# Autodesk Inventor assembly: joint4
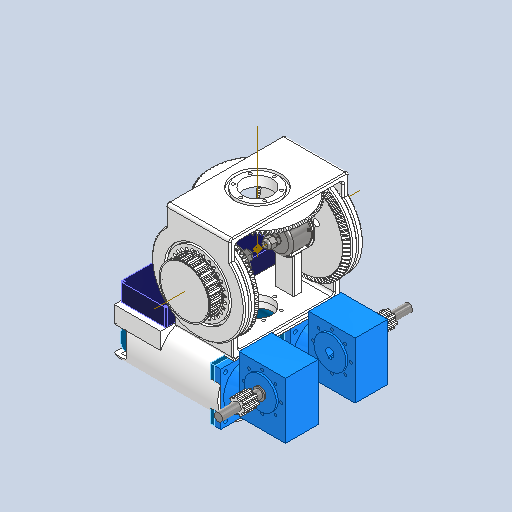
[picture p0: Inventor's stored thumbnail of the model, 512x512]
Saved by Autodesk Inventor 2025.3 (Build 293356030, 356C)
## iProperties
Created: 2025-08-31
Part Number: joint4
Document SubType Name: Assembly
Designer: MSI
Mass: 16930.7 g
Surface Area: 10614.2 cm^2
Volume: 6203.06 cm^3
Density: 2.72942 g/cm^3
Author: MSI
## Documents named in this file (15)
- C:\Users\MSI\Desktop\Project\11. 로봇팔\Robot Arm Model\Robot_Arm_6_v1\joint3.iam
- C:\Users\MSI\Desktop\Project\11. 로봇팔\Robot Arm Model\Robot_Arm_6_v1\motor_holder_1.ipt
- C:\Users\MSI\Desktop\Project\11. 로봇팔\Robot Arm Model\Robot_Arm_6_v1\NMRV30_motor.iam
- C:\Users\MSI\Desktop\Project\11. 로봇팔\Robot Arm Model\Robot_Arm_6_v1\base.ipt
- C:\Users\MSI\Desktop\Project\11. 로봇팔\Robot Arm Model\Robot_Arm_6_v1\frame.ipt
- C:\Users\MSI\Desktop\Project\11. 로봇팔\Robot Arm Model\Robot_Arm_6_v1\miter_gear_center.ipt
- C:\Users\MSI\Desktop\Project\11. 로봇팔\Robot Arm Model\Robot_Arm_6_v1\encoder.ipt
- C:\Users\MSI\Desktop\Project\11. 로봇팔\Robot Arm Model\Robot_Arm_6_v1\belt_pulley_1.ipt
- C:\Users\MSI\Desktop\Project\11. 로봇팔\Robot Arm Model\Robot_Arm_6_v1\belt_pulley_2.ipt
- C:\Users\MSI\Desktop\Project\11. 로봇팔\Robot Arm Model\Robot_Arm_6_v1\motor_shaft.ipt
- C:\Users\MSI\Desktop\Project\11. 로봇팔\Robot Arm Model\Robot_Arm_6_v1\motor_driver.ipt
- C:\Users\MSI\Desktop\Project\11. 로봇팔\Robot Arm Model\Robot_Arm_6_v1\joint3_meteor.iam
- C:\Users\MSI\Desktop\Project\11. 로봇팔\Robot Arm Model\Robot_Arm_6_v1\encoder_frame.ipt
- C:\Users\MSI\Desktop\Project\11. 로봇팔\Robot Arm Model\Robot_Arm_6_v1\miter_gear_left_axis.ipt
- C:\Users\MSI\Desktop\Project\11. 로봇팔\Robot Arm Model\Robot_Arm_6_v1\miter_gear_right_axis.ipt
## Components (22 placed, 13 different names)
1. base:1 — 회전:1, 강체:5, 강체:17, 강체:19
2. frame:1 — 회전:1, 회전:4
3. 베벨 기어2:1 — 회전:4
4. 베벨 기어1:3 — 강체:20
5. 베벨 기어1:4 — 강체:21
6. encoder:1 — 강체:18
7. encoder:2 — 강체:16
8. NMRV30_motor:1 [sub-assembly] — 강체:3, 강체:9, 강체:11
9. NMRV30_motor:2 [sub-assembly] — 강체:4, 강체:7, 강체:10
10. motor_holder_1:1 — 강체:3, 강체:4, 강체:5, 강체:12, 강체:13
11. 동기식 풀리1:1 — 강체:7
12. 동기식 풀리2:1 — 강체:6
13. 동기식 풀리1:2 — 강체:9
14. 동기식 풀리2:2 — 강체:8
15. motor_shaft:1 — 강체:11
16. motor_shaft:2 — 강체:10
17. motor_driver:1 — 강체:13
18. motor_driver:2 — 강체:12
19. joint3_meteor:1 [sub-assembly] — 강체:6, 강체:20
20. joint3_meteor:2 [sub-assembly] — 강체:8, 강체:21
21. encoder_frame:1 — 강체:16, 강체:17
22. encoder_frame:2 — 강체:18, 강체:19
## Relationships (19: WeldJoint 17, RevoluteJoint 2)
- 회전:1 [RevoluteJoint]: base:1 ↔ frame:1
- 회전:4 [RevoluteJoint]: frame:1 ↔ 베벨 기어2:1
- 강체:18 [WeldJoint]: encoder:1 ↔ encoder_frame:2
- 강체:16 [WeldJoint]: encoder:2 ↔ encoder_frame:1
- 강체:3 [WeldJoint]: NMRV30_motor:1 ↔ motor_holder_1:1
- 강체:4 [WeldJoint]: NMRV30_motor:2 ↔ motor_holder_1:1
- 강체:5 [WeldJoint]: base:1 ↔ motor_holder_1:1
- 강체:6 [WeldJoint]: 동기식 풀리2:1 ↔ joint3_meteor:1
- 강체:7 [WeldJoint] (15 mm): NMRV30_motor:2 ↔ 동기식 풀리1:1
- 강체:8 [WeldJoint]: 동기식 풀리2:2 ↔ joint3_meteor:2
- 강체:9 [WeldJoint] (15 mm): NMRV30_motor:1 ↔ 동기식 풀리1:2
- 강체:10 [WeldJoint]: NMRV30_motor:2 ↔ motor_shaft:2
- 강체:11 [WeldJoint]: NMRV30_motor:1 ↔ motor_shaft:1
- 강체:12 [WeldJoint]: motor_holder_1:1 ↔ motor_driver:2
- 강체:13 [WeldJoint]: motor_holder_1:1 ↔ motor_driver:1
- 강체:17 [WeldJoint]: base:1 ↔ encoder_frame:1
- 강체:19 [WeldJoint]: base:1 ↔ encoder_frame:2
- 강체:20 [WeldJoint]: 베벨 기어1:3 ↔ joint3_meteor:1
- 강체:21 [WeldJoint]: 베벨 기어1:4 ↔ joint3_meteor:2
